# Autodesk Inventor assembly: 48452cx1
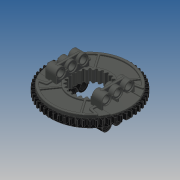
[picture p0: Inventor's stored thumbnail of the model, 180x180]
Saved by Autodesk Inventor 2022.2 (Build 262287000, 287)
## iProperties
Created: 2015-01-10
Part Number: 48452cx1
Document SubType Name: Assembly
Designer: D. Kohfeld
Mass: 12.2298 g
Surface Area: 171.436 cm^2
Volume: 11.5375 cm^3
Density: 1.06 g/cm^3
Description: Technic, Gear 56
Author: D. Kohfeld
## Documents named in this file (3)
- D:\Inventor\Projekte\Muther\LEGO Technic\LEGO Pieces\48452cx1-DkBluishGray.iam
- D:\Inventor\Projekte\Muther\LEGO Technic\LEGO Pieces\Einzelteile zu Baugruppen\48168-Black.ipt
- D:\Inventor\Projekte\Muther\LEGO Technic\LEGO Pieces\Einzelteile zu Baugruppen\48452-DkBluishGray.ipt
## Components (2 placed, 2 different names)
1. 48452-DkBluishGray:1 — Insert:1
2. 48168-Black:1 — Insert:1
## Relationships (1: Insert 1)
- Insert:1: 48452-DkBluishGray:1 ↔ 48168-Black:1
